# Autodesk Inventor assembly: Assembly1
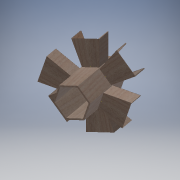
[picture p0: Inventor's stored thumbnail of the model, 180x180]
Saved by Autodesk Inventor 2017 (Build 210142000, 142)
## iProperties
Created: 2016-07-03
Part Number: Assembly1
Document SubType Name: Assembly
Designer: Ing
Author: Ing
## Documents named in this file (3)
- C:\Users\Ing\Dropbox\DACK Chile\Mesa\Assembly1.iam
- C:\Users\Ing\Dropbox\DACK Chile\Mesa\Hexagono.ipt
- C:\Users\Ing\Dropbox\DACK Chile\Mesa\Modulo.ipt
## Components (7 placed, 2 different names)
1. Hexagono:1 — Slider:1, Slider:2, Slider:3, Slider:4, Slider:5, Slider:6
2. Modulo:1 — Slider:1
3. Modulo:2 — Slider:2
4. Modulo:3 — Slider:3
5. Modulo:4 — Slider:4
6. Modulo:5 — Slider:5
7. Modulo:6 — Slider:6
## Relationships (6: TranslationJoint 6)
- Slider:1 [TranslationJoint]: Hexagono:1 ↔ Modulo:1
- Slider:2 [TranslationJoint]: Hexagono:1 ↔ Modulo:2
- Slider:3 [TranslationJoint]: Hexagono:1 ↔ Modulo:3
- Slider:4 [TranslationJoint]: Hexagono:1 ↔ Modulo:4
- Slider:5 [TranslationJoint]: Hexagono:1 ↔ Modulo:5
- Slider:6 [TranslationJoint]: Hexagono:1 ↔ Modulo:6
